# Autodesk Inventor assembly: Leg_joint_roll
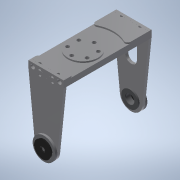
[picture p0: Inventor's stored thumbnail of the model, 180x180]
Saved by Autodesk Inventor 2020.4 (Build 244396000, 396)
## iProperties
Created: 2016-05-01
Part Number: Leg_joint_roll
Document SubType Name: Assembly
Designer: hiroaki
Mass: 101.489 g
Surface Area: 218.083 cm^2
Volume: 17.9148 cm^3
Density: 5.6651 g/cm^3
Author: hiroaki
## Documents named in this file (7)
- C:\Users\Masato\Documents\Inventor\CIT Brains_Inventor\OpenPlatform_ver3_0\LowerBody\Leg_joint_roll\Leg_Joint_roll.iam
- C:\Users\Masato\Documents\Inventor\CIT Brains_Inventor\OpenPlatform_ver3_0\LowerBody\Leg_joint_roll\Leg_Joint_roll_vertical_back.ipt
- C:\Users\Masato\Documents\Inventor\CIT Brains_Inventor\OpenPlatform_ver3_0\LowerBody\Leg_joint_roll\Leg_Joint_roll_vertical_front.ipt
- C:\Users\Masato\Documents\Inventor\CIT Brains_Inventor\OpenPlatform_ver3_0\Ready_Made\UUW-0312-10BH.ipt
- C:\Users\Masato\Documents\Inventor\CIT Brains_Inventor\OpenPlatform_ver3_0\Ready_Made\80F-0603.ipt
- C:\Users\Masato\Documents\Inventor\CIT Brains_Inventor\OpenPlatform_ver3_0\Ready_Made\LFW-0815.ipt
- C:\Users\Masato\Documents\Inventor\CIT Brains_Inventor\OpenPlatform_ver3_0\LowerBody\Leg_joit\Leg_joint_basis_frame.ipt
## Components (9 placed, 6 different names)
1. Leg_Joint_roll_vertical_back:1 — 挿入:42, 挿入:47, 挿入:51, 挿入:52
2. Leg_Joint_roll_vertical_front:1 — 挿入:43, 挿入:46, 挿入:49, 挿入:50
3. UUW-0312-10BH:3 — 挿入:45
4. UUW-0312-10BH:4 — 挿入:48
5. 80F-0603:1 — 挿入:43
6. 80F-0603:2 — 挿入:42
7. LFW-0815:1 — 挿入:45, 挿入:46
8. LFW-0815:2 — 挿入:47, 挿入:48
9. Leg_joint_basis_frame:1 — 挿入:49, 挿入:50, 挿入:51, 挿入:52
## Relationships (10: Insert 10)
- 挿入:42 [Insert]: Leg_Joint_roll_vertical_back:1 ↔ 80F-0603:2
- 挿入:43 [Insert]: Leg_Joint_roll_vertical_front:1 ↔ 80F-0603:1
- 挿入:45 [Insert]: UUW-0312-10BH:3 ↔ LFW-0815:1
- 挿入:46 [Insert]: Leg_Joint_roll_vertical_front:1 ↔ LFW-0815:1
- 挿入:47 [Insert]: Leg_Joint_roll_vertical_back:1 ↔ LFW-0815:2
- 挿入:48 [Insert]: UUW-0312-10BH:4 ↔ LFW-0815:2
- 挿入:49 [Insert]: Leg_Joint_roll_vertical_front:1 ↔ Leg_joint_basis_frame:1
- 挿入:50 [Insert]: Leg_Joint_roll_vertical_front:1 ↔ Leg_joint_basis_frame:1
- 挿入:51 [Insert]: Leg_Joint_roll_vertical_back:1 ↔ Leg_joint_basis_frame:1
- 挿入:52 [Insert]: Leg_Joint_roll_vertical_back:1 ↔ Leg_joint_basis_frame:1
